# Autodesk Inventor assembly: Teensy3.6 with header pins
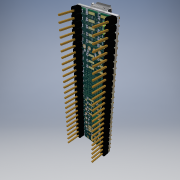
[picture p0: Inventor's stored thumbnail of the model, 180x180]
Saved by Autodesk Inventor 2016 (Build 200138000, 138)
## iProperties
Created: 2014-04-23
Part Number: Teensy3.6 with header pins
Document SubType Name: Assembly
Designer: larraguetajunior
Description: Teensy3.1/3.2
Mass: 3 g
Surface Area: 27.9252 cm^2
Volume: 1.41306 cm^3
Author: JLJ
## Documents named in this file (5)
- D:\cloud\Dropbox\UAV\- Air Data Computer\Asgard\Off the shelf\teensy3.6\Teensy3.6withheaders.iam
- D:\cloud\Dropbox\UAV\- Air Data Computer\Asgard\Off the shelf\teensy3.6\Teensyboard.ipt
- D:\cloud\Dropbox\UAV\- Air Data Computer\Asgard\Off the shelf\teensy3.6\MiniUSB.ipt
- D:\cloud\Dropbox\UAV\- Air Data Computer\Asgard\Off the shelf\Connectors\24 Pin Straight Header.iam
- D:\cloud\Dropbox\UAV\- Air Data Computer\Asgard\Off the shelf\MICRO SD ADAPTER\5031821852MICROSDADAPTER.ipt
## Components (5 placed, 4 different names)
1. 101 Teensyboard:1 — Allineato:3, Allineato:2, Flush:5, Coincidente:4, Allineato:4, Mate:7, Angle:1, Rigid:1, Mate:8
2. MiniUSB:1 — Flush:5, Coincidente:4
3. 5031821852MICROSDADAPTER:1 — Mate:8
4. 24 Pin Straight Header:1 [sub-assembly] — Mate:7, Angle:1, Rigid:1
5. 24 Pin Straight Header:2 [sub-assembly]
## Component patterns: (2 elements, first: 24 Pin Straight Header:1)
## Relationships (9: Flush 4, Mate 3, Angle 1, WeldJoint 1)
- Allineato:3 [Flush]: 101 Teensyboard:1
- Allineato:2 [Flush]: 101 Teensyboard:1
- Flush:5: 101 Teensyboard:1 ↔ MiniUSB:1
- Coincidente:4 [Mate]: 101 Teensyboard:1 ↔ MiniUSB:1
- Allineato:4 [Flush]: 101 Teensyboard:1
- Mate:7: 101 Teensyboard:1 ↔ 24 Pin Straight Header:1
- Angle:1 (0 deg): 101 Teensyboard:1 ↔ 24 Pin Straight Header:1
- Rigid:1 [WeldJoint]: 101 Teensyboard:1 ↔ 24 Pin Straight Header:1
- Mate:8: 101 Teensyboard:1 ↔ 5031821852MICROSDADAPTER:1
